# Autodesk Inventor assembly: Leg_Frame_Connector_16mm_MIR1
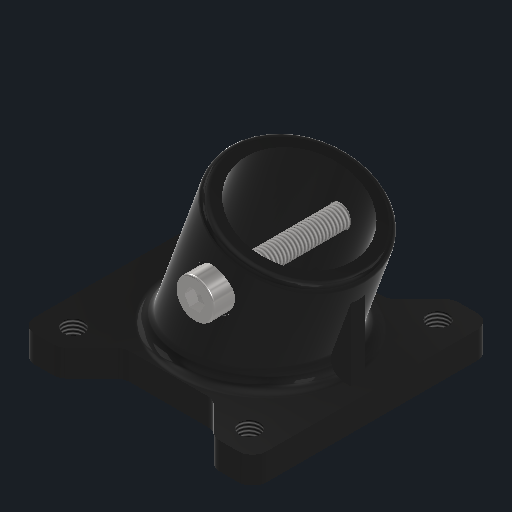
[picture p0: Inventor's stored thumbnail of the model, 512x512]
Saved by Autodesk Inventor 2024.1 (Build 281209000, 209)
## iProperties
Created: 2023-12-04
Part Number: Leg_Frame_Connector_16mm_MIR1
Document SubType Name: Assembly
Designer: dzw04
Author: dzw04
## Documents named in this file (4)
- C:\Users\dzw04\Saxion\Mechatronica Lectoraat LMECH LED - Database ARG\Component_Database\SARAX\01. CAD\01. 3D_Drawing\02. Sub_Assemblies\Landing_Gear\02. Sub_Assemblies\Leg_Frame_Connector_16mm_MIR1.iam
- C:\Users\dzw04\Saxion\Mechatronica Lectoraat LMECH LED - Database ARG\Component_Database\SARAX\01. CAD\01. 3D_Drawing\02. Sub_Assemblies\Landing_Gear\01. Parts\Leg_Frame_Connector_16mm_MIR1.ipt
- C:\Users\dzw04\OneDrive - Saxion\Documenten\Inventor\Content Center Files\R2024\en-US\ISO 4762(2)\ISO 4762 - M3 x 20ISO.ipt
- C:\Users\dzw04\OneDrive - Saxion\Documenten\Inventor\Content Center Files\R2024\en-US\ISO 4035(2)\ISO 4035 - M3 - ISO.ipt
## Components (3 placed, 3 different names)
1. Leg_Frame_Connector_16mm_MIR1:1 — Mate:2, Mate:1, Mate:4, Mate:3
2. ISO 4762 M3 x 20:1 — Mate:2, Mate:1
3. ISO 4035 M3:1 — Mate:4, Mate:3
## Relationships (4: Mate 4)
- Mate:2: Leg_Frame_Connector_16mm_MIR1:1 ↔ ISO 4762 M3 x 20:1
- Mate:1: Leg_Frame_Connector_16mm_MIR1:1 ↔ ISO 4762 M3 x 20:1
- Mate:4: Leg_Frame_Connector_16mm_MIR1:1 ↔ ISO 4035 M3:1
- Mate:3: Leg_Frame_Connector_16mm_MIR1:1 ↔ ISO 4035 M3:1
